# Autodesk Inventor assembly: Assembly1
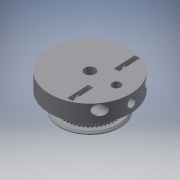
[picture p0: Inventor's stored thumbnail of the model, 180x180]
Saved by Autodesk Inventor 2018 (Build 220112000, 112)
## iProperties
Created: 2018-07-04
Part Number: Assembly1
Document SubType Name: Assembly
Designer: Cole Tucker
Author: Cole Tucker
## Documents named in this file (3)
- C:\Users\Cole Tucker\OneDrive\FRC-mxpProject\Cad\sweepSensor\Inventor\v2\Assembly1.iam
- C:\Users\Cole Tucker\Downloads\SDP_a_6d51m048df0606.ipt
- C:\Users\Cole Tucker\OneDrive\FRC-mxpProject\Cad\sweepSensor\Inventor\v2\table.ipt
## Components (2 placed, 2 different names)
1. SDP_a_6d51m048df0606:1 — Mate:1, Mate:2
2. table:1 — Mate:1, Mate:2
## Relationships (2: Mate 2)
- Mate:1: SDP_a_6d51m048df0606:1 ↔ table:1
- Mate:2: SDP_a_6d51m048df0606:1 ↔ table:1
